# Autodesk Inventor assembly: EngranajesParte
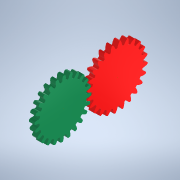
[picture p0: Inventor's stored thumbnail of the model, 180x180]
Saved by Autodesk Inventor 2020.3 (Build 243373000, 373)
## iProperties
Created: 2020-07-27
Part Number: EngranajesParte
Document SubType Name: Assembly
Designer: juanp
Author: juanp
## Documents named in this file (3)
- C:\Users\juanp\Desktop\Extr\EngranajesParte.iam
- C:\Users\juanp\Desktop\Extr\Engranaje A.ipt
- C:\Users\juanp\Desktop\Extr\Engranaje B.ipt
## Components (2 placed, 2 different names)
1. Engranaje A:1 — Flush:2, Mate:2, Mate:3, Flush:3, Mate:5, Angle:2
2. Engranaje B:1 — Flush:2, Mate:2, Mate:4, Angle:1
## Relationships (8: Mate 4, Flush 2, Angle 2)
- Flush:2: Engranaje A:1 ↔ Engranaje B:1
- Mate:2 (49.41 mm): Engranaje A:1 ↔ Engranaje B:1
- Mate:3: Engranaje A:1
- Mate:4: Engranaje B:1
- Flush:3: Engranaje A:1
- Mate:5: Engranaje A:1
- Angle:1 (-1000 deg): Engranaje B:1
- Angle:2 (1000 deg): Engranaje A:1
